# Autodesk Inventor assembly: mouse
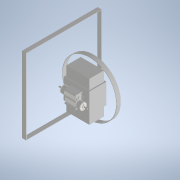
[picture p0: Inventor's stored thumbnail of the model, 180x180]
Saved by Autodesk Inventor 2020 (Build 240168000, 168)
## iProperties
Created: 2020-03-14
Part Number: mouse
Document SubType Name: Assembly
Designer: atmat
Author: atmat
## Documents named in this file (6)
- D:\1.Projects\1.Roboty\5. Micromouse\Czesci\mouse.iam
- D:\1.Projects\1.Roboty\2.JadeJager\Czesci\Ver 1\Motor.ipt
- D:\1.Projects\1.Roboty\5. Micromouse\Czesci\Koszyk.ipt
- D:\1.Projects\1.Roboty\5. Micromouse\Czesci\Main.ipt
- D:\1.Projects\1.Roboty\5. Micromouse\Czesci\czujka.ipt
- D:\1.Projects\1.Roboty\5. Micromouse\Czesci\frame.ipt
## Components (6 placed, 5 different names)
1. Motor:1 — Mate:5, Tangent:2, Mate:6
2. Motor:2 — Mate:3, Tangent:1, Mate:7
3. Koszyk:1 — Mate:1, Mate:2, Mate:3, Tangent:1, Mate:4, Mate:5, Tangent:2, Mate:6, Mate:7, Mate:8, Mate:9, Mate:11, Flush:1
4. Main:1 — Mate:8, Mate:9, Mate:10
5. czujka:1 — Mate:11, Flush:1
6. frame:1
## Relationships (14: Mate 11, Tangent 2, Flush 1)
- Mate:1: Koszyk:1
- Mate:2 (-31 mm): Koszyk:1
- Mate:3: Motor:2 ↔ Koszyk:1
- Tangent:1: Motor:2 ↔ Koszyk:1
- Mate:4 (-24.5 mm): Koszyk:1
- Mate:5: Motor:1 ↔ Koszyk:1
- Tangent:2: Motor:1 ↔ Koszyk:1
- Mate:6: Motor:1 ↔ Koszyk:1
- Mate:7: Motor:2 ↔ Koszyk:1
- Mate:8: Koszyk:1 ↔ Main:1
- Mate:9: Koszyk:1 ↔ Main:1
- Mate:10 (-48 mm): Main:1
- Mate:11: Koszyk:1 ↔ czujka:1
- Flush:1: Koszyk:1 ↔ czujka:1
